# Autodesk Inventor assembly: Model-1
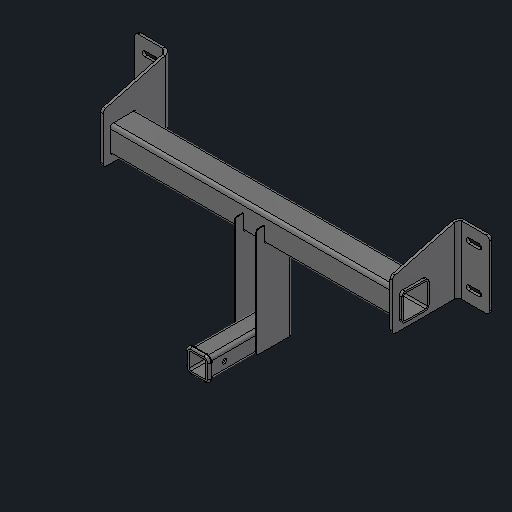
[picture p0: Inventor's stored thumbnail of the model, 512x512]
Saved by Autodesk Inventor 2025.1 (Build 291241000, 241)
## iProperties
Created: 2026-02-13
Part Number: Model-1
Document SubType Name: Assembly
Designer: Desktop -24
encoded128: ÌStandard (in)rÎ
Family: ASSEMBLY
Author: Desktop -24
## Documents named in this file (6)
- F:\OneDrive - nLeague Technologies Private Limited\Desktop\Sharath Chandra\Rear Hitch\Model-1\Model-1.iam
- F:\OneDrive - nLeague Technologies Private Limited\Desktop\Sharath Chandra\Rear Hitch\Model-1\Model-1_Base Tube-1.ipt
- F:\OneDrive - nLeague Technologies Private Limited\Desktop\Sharath Chandra\Rear Hitch\Model-1\Model-1_Base Tube-3.ipt
- F:\OneDrive - nLeague Technologies Private Limited\Desktop\Sharath Chandra\Rear Hitch\Model-1\Model-1_Base Sheet.ipt
- F:\OneDrive - nLeague Technologies Private Limited\Desktop\Sharath Chandra\Rear Hitch\Model-1\Model-1_Sheet-LH.ipt
- F:\OneDrive - nLeague Technologies Private Limited\Desktop\Sharath Chandra\Rear Hitch\Model-1\Model-1_Sheet-RH.ipt
## Components (5 placed, 5 different names)
1. Model-1_Base Tube-1:1 — Mate:1, Mate:6, Mate:3, Flush:2, Flush:5, Mate:8, Mate:9, Flush:6, Mate:10, Mate:11
2. Model-1_Base Tube-3:1 — Flush:1, Flush:4, Mate:7
3. Model-1_Sheet-LH:1 — Flush:5, Mate:8, Mate:9
4. Model-1_Base Sheet:1 — Mate:1, Mate:6, Flush:1, Flush:2, Flush:4, Mate:7
5. Model-1_Sheet-RH:1 — Flush:6, Mate:10, Mate:11
## Relationships (13: Mate 8, Flush 5)
- Mate:1: Model-1_Base Tube-1:1 ↔ Model-1_Base Sheet:1
- Mate:6: Model-1_Base Tube-1:1 ↔ Model-1_Base Sheet:1
- Mate:3: Model-1_Base Tube-1:1
- Flush:1: Model-1_Base Tube-3:1 ↔ Model-1_Base Sheet:1
- Flush:2: Model-1_Base Tube-1:1 ↔ Model-1_Base Sheet:1
- Flush:4: Model-1_Base Tube-3:1 ↔ Model-1_Base Sheet:1
- Mate:7: Model-1_Base Tube-3:1 ↔ Model-1_Base Sheet:1
- Flush:5 (9.525 mm): Model-1_Base Tube-1:1 ↔ Model-1_Sheet-LH:1
- Mate:8: Model-1_Base Tube-1:1 ↔ Model-1_Sheet-LH:1
- Mate:9: Model-1_Base Tube-1:1 ↔ Model-1_Sheet-LH:1
- Flush:6 (-9.525 mm): Model-1_Base Tube-1:1 ↔ Model-1_Sheet-RH:1
- Mate:10: Model-1_Base Tube-1:1 ↔ Model-1_Sheet-RH:1
- Mate:11: Model-1_Base Tube-1:1 ↔ Model-1_Sheet-RH:1
